# Autodesk Inventor assembly: Assembly Exploded
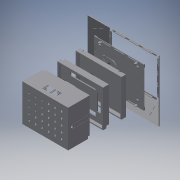
[picture p0: Inventor's stored thumbnail of the model, 180x180]
Saved by Autodesk Inventor 2017 (Build 210142000, 142)
## iProperties
Created: 2018-02-08
Part Number: Assembly Exploded
Document SubType Name: Assembly
Designer: Arjuna
Author: Arjuna
## Documents named in this file (6)
- D:\Users\Arjuna\Documents\NTU\FYP\Hardware\Assembly Exploded.iam
- D:\Users\Arjuna\Documents\NTU\FYP\Hardware\Bottom Roof.ipt
- D:\Users\Arjuna\Documents\NTU\FYP\Hardware\Bottom Assembly.iam
- D:\Users\Arjuna\Documents\NTU\FYP\Hardware\Platform Assembly.iam
- D:\Users\Arjuna\Documents\NTU\FYP\Hardware\Top Roof Assembly.iam
- D:\Users\Arjuna\Documents\NTU\FYP\Hardware\Roof Extension Assembly.iam
## Components (5 placed, 5 different names)
1. Bottom Assembly:1 [sub-assembly] — Flush:1, Flush:2, Flush:3, Flush:4, Flush:5, Flush:6, Flush:7, Flush:8, Flush:9, Mate:1
2. Platform Assembly:1 [sub-assembly] — Flush:4, Flush:5, Mate:1, Mate:2
3. Bottom Roof:1 — Flush:6, Flush:7, Mate:2, Mate:3
4. Top Roof Assembly:1 [sub-assembly] — Flush:8, Flush:9, Mate:3, Mate:4
5. Roof Extension Assembly:1 [sub-assembly] — Flush:10, Flush:11, Mate:4
## Relationships (15: Flush 11, Mate 4)
- Flush:1: Bottom Assembly:1
- Flush:2: Bottom Assembly:1
- Flush:3: Bottom Assembly:1
- Flush:4: Bottom Assembly:1 ↔ Platform Assembly:1
- Flush:5: Bottom Assembly:1 ↔ Platform Assembly:1
- Flush:6: Bottom Assembly:1 ↔ Bottom Roof:1
- Flush:7: Bottom Assembly:1 ↔ Bottom Roof:1
- Flush:8: Bottom Assembly:1 ↔ Top Roof Assembly:1
- Flush:9: Bottom Assembly:1 ↔ Top Roof Assembly:1
- Mate:1 (75 mm): Bottom Assembly:1 ↔ Platform Assembly:1
- Mate:2 (75 mm): Platform Assembly:1 ↔ Bottom Roof:1
- Mate:3 (75 mm): Bottom Roof:1 ↔ Top Roof Assembly:1
- Flush:10: Roof Extension Assembly:1
- Flush:11: Roof Extension Assembly:1
- Mate:4 (75 mm): Top Roof Assembly:1 ↔ Roof Extension Assembly:1
